# Autodesk Inventor assembly: SACMI DPA TILES GRIP
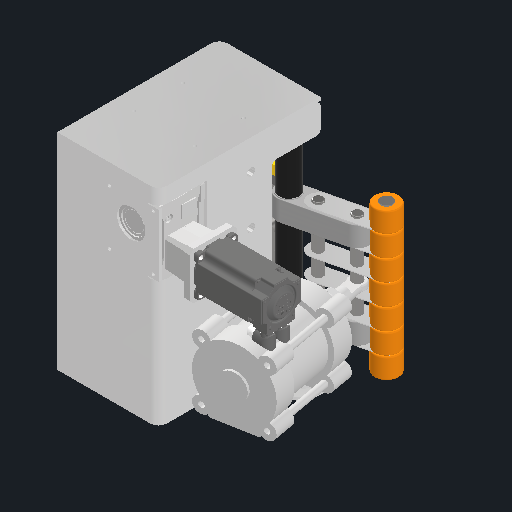
[picture p0: Inventor's stored thumbnail of the model, 512x512]
Saved by Autodesk Inventor 2025 (Build 290162000, 162)
## iProperties
Created: 2024-05-26
Part Number: SACMI DPA TILES GRIP
Document SubType Name: Assembly
Designer: zulet
Author: zulet
## Documents named in this file (7)
- D:\UNAL\2024-1S\APM\Digital Factory\Packaging Machine\SACMI DPA TILES GRIP.iam
- D:\UNAL\2024-1S\APM\Digital Factory\Packaging Machine\SACMI DPA TILES GRIP BASE.ipt
- D:\UNAL\2024-1S\APM\Digital Factory\Linear Guides & Ball Screws\guidage_lineaire_shs55_lv_1_ss___492l_66.iam
- D:\UNAL\2024-1S\APM\Digital Factory\Packaging Machine\Assembly2.iam
- D:\UNAL\2024-1S\APM\Digital Factory\Packaging Machine\TILES GRIP ROLLERS.ipt
- D:\UNAL\2024-1S\APM\Digital Factory\Pneumatic Cylinders and Guides\cylinder_452500010050_010754_0.iam
- D:\UNAL\2024-1S\APM\Digital Factory\Pneumatic Cylinders and Guides\cylinder_45001223510555_0.iam
## Components (6 placed, 6 different names)
1. SACMI DPA TILES GRIP BASE:1 — Rigid:2, Rigid:3, Cylindrical:1, Rotational:1
2. guidage_lineaire_shs55_lv_1_ss___492l_66:1 [sub-assembly] — Rigid:3, Rigid:4
3. Assembly2:1 [sub-assembly] — Rigid:2
4. TILES GRIP ROLLERS:1 — Cylindrical:1, Cylindrical:2
5. cylinder_452500010050_010754_0:1 [sub-assembly] — Rigid:4
6. cylinder_45001223510555_0:1 [sub-assembly] — Rotational:1, Cylindrical:2
## Relationships (6: WeldJoint 3, CylindricalJoint 2, RevoluteJoint 1)
- Rigid:2 [WeldJoint]: SACMI DPA TILES GRIP BASE:1 ↔ Assembly2:1
- Rigid:3 [WeldJoint]: SACMI DPA TILES GRIP BASE:1 ↔ guidage_lineaire_shs55_lv_1_ss___492l_66:1
- Rigid:4 [WeldJoint]: guidage_lineaire_shs55_lv_1_ss___492l_66:1 ↔ cylinder_452500010050_010754_0:1
- Cylindrical:1: SACMI DPA TILES GRIP BASE:1 ↔ TILES GRIP ROLLERS:1
- Rotational:1 [RevoluteJoint]: SACMI DPA TILES GRIP BASE:1 ↔ cylinder_45001223510555_0:1
- Cylindrical:2: TILES GRIP ROLLERS:1 ↔ cylinder_45001223510555_0:1
